# Autodesk Inventor assembly: palp-boron-hybrid
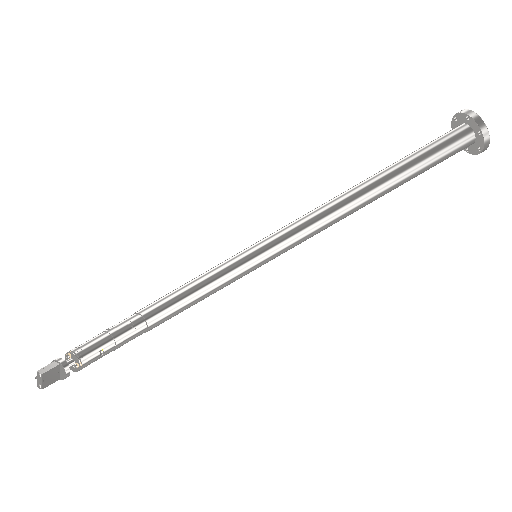
[picture p0: Inventor's stored thumbnail of the model, 512x512]
Saved by Autodesk Inventor 2026.2 (Build 302298000, 298)
## iProperties
Created: 2024-05-30
Part Number: palp-boron-hybrid
Document SubType Name: Assembly
Designer: kuzmin
Author: kuzmin
## Documents named in this file (10)
- D:\repos\PIHTI\BoronProbe\palp-boron-hybrid.iam
- D:\repos\PIHTI\PALP\Prototype-PALP-ring-to-pipe-adapter_4mm.ipt
- D:\repos\PIHTI\ContentCenter\Ceramics\Electric-feeds\feed_4.ipt
- D:\repos\PIHTI\PALP\Prototype-PALP-pipe-neck-straight.ipt
- D:\repos\PIHTI\PALP\Prototype-PALP-CF34-flange.ipt
- D:\repos\PIHTI\PALP\Prototype-PALP-34pipe-with-flange.iam
- D:\repos\PIHTI\PALP\wire_connector.ipt
- D:\repos\PIHTI\BoronProbe\BoronHead.iam
- D:\repos\PIHTI\SpectroscopySystem_Hayashi\Probe\clamp_L58.iam
- D:\repos\PIHTI\SpectroscopySystem_Hayashi\Probe\clamp_L50.iam
## Components (13 placed, 9 different names)
1. Prototype-PALP-34pipe-with-flange:1 [sub-assembly]
2. Prototype-PALP-ring-to-pipe-adapter_4mm:1 — 回転:6, フラッシュ:1, リジッド:7, リジッド:8
3. feed_4:1 — 円柱状:1, リジッド:8
4. feed_4:2 — 円柱状:2, リジッド:7
5. Prototype-PALP-pipe-neck-straight:1 — 回転:6, リジッド:4, メイト:11, メイト:12
6. Prototype-PALP-CF34-flange:1 — リジッド:4, メイト:5, リジッド:9, メイト:14
7. wire_connector:1 — 円柱状:1
8. wire_connector:2 — 円柱状:2
9. BoronHead:1 [sub-assembly] — リジッド:9, メイト:6, メイト:7, メイト:10
10. clamp_L58:1 [sub-assembly] — メイト:6, メイト:8, メイト:9, フラッシュ:2, メイト:10
11. clamp_L58:2 [sub-assembly] — メイト:7, メイト:8, メイト:9, フラッシュ:2
12. clamp_L50:1 [sub-assembly] — メイト:11, メイト:13, フラッシュ:3
13. clamp_L50:2 [sub-assembly] — メイト:12, メイト:13, フラッシュ:3, メイト:14
## Relationships (22: Mate 11, WeldJoint 4, Flush 3, RevoluteJoint 2, CylindricalJoint 2)
- [Mate]: Prototype-PALP-34pipe-with-flange:1 ↔ Prototype-PALP-ring-to-pipe-adapter_4mm:1
- [RevoluteJoint]: Prototype-PALP-34pipe-with-flange:1 ↔ Prototype-PALP-ring-to-pipe-adapter_4mm:1
- 回転:6 [RevoluteJoint]: Prototype-PALP-ring-to-pipe-adapter_4mm:1 ↔ Prototype-PALP-pipe-neck-straight:1
- リジッド:4 [WeldJoint]: Prototype-PALP-pipe-neck-straight:1 ↔ Prototype-PALP-CF34-flange:1
- フラッシュ:1 [Flush]: Prototype-PALP-ring-to-pipe-adapter_4mm:1
- メイト:5 [Mate]: Prototype-PALP-CF34-flange:1
- 円柱状:1 [CylindricalJoint]: feed_4:1 ↔ wire_connector:1
- 円柱状:2 [CylindricalJoint]: feed_4:2 ↔ wire_connector:2
- リジッド:7 [WeldJoint]: Prototype-PALP-ring-to-pipe-adapter_4mm:1 ↔ feed_4:2
- リジッド:8 [WeldJoint]: Prototype-PALP-ring-to-pipe-adapter_4mm:1 ↔ feed_4:1
- リジッド:9 [WeldJoint]: Prototype-PALP-CF34-flange:1 ↔ BoronHead:1
- メイト:6 [Mate]: BoronHead:1 ↔ clamp_L58:1
- メイト:7 [Mate]: BoronHead:1 ↔ clamp_L58:2
- メイト:8 [Mate]: clamp_L58:1 ↔ clamp_L58:2
- メイト:9 [Mate]: clamp_L58:1 ↔ clamp_L58:2
- フラッシュ:2 [Flush]: clamp_L58:1 ↔ clamp_L58:2
- メイト:10 [Mate] (0.5 mm): BoronHead:1 ↔ clamp_L58:1
- メイト:11 [Mate]: Prototype-PALP-pipe-neck-straight:1 ↔ clamp_L50:1
- メイト:12 [Mate]: Prototype-PALP-pipe-neck-straight:1 ↔ clamp_L50:2
- メイト:13 [Mate]: clamp_L50:1 ↔ clamp_L50:2
- フラッシュ:3 [Flush]: clamp_L50:1 ↔ clamp_L50:2
- メイト:14 [Mate] (0.5 mm): Prototype-PALP-CF34-flange:1 ↔ clamp_L50:2
